# Autodesk Inventor assembly: MotorAssembly0
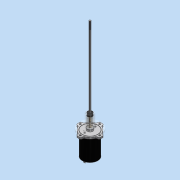
[picture p0: Inventor's stored thumbnail of the model, 180x180]
Saved by Autodesk Inventor 2017.3 (Build 213256000, 256)
## iProperties
Created: 2016-10-13
Part Number: MotorAssembly0
Document SubType Name: Assembly
Designer: techn
Author: techn
## Documents named in this file (7)
- G:\Projects\Submarine\Submarine-project\CAD\aft\MotorAssembly0.iam
- G:\Projects\Submarine\Submarine-project\CAD\aft\ShaftSeal\4mmShaftSeal.iam
- G:\Projects\Submarine\Submarine-project\CAD\aft\540DCMotor.ipt
- G:\Projects\Submarine\Submarine-project\CAD\aft\MotorMount.ipt
- G:\Projects\Submarine\Submarine-project\CAD\aft\MotorShaftCoupler.ipt
- G:\Projects\Submarine\Submarine-project\CAD\aft\DriveShaft4mm.ipt
- G:\Projects\Submarine\Submarine-project\CAD\aft\MotorMountNutHolder.ipt
## Components (6 placed, 6 different names)
1. 4mmShaftSeal:1 [sub-assembly] — Mate:3, Flush:1, Mate:7
2. 540DCMotor:1 — Mate:1, Mate:2, Mate:3, Mate:4, Mate:6
3. MotorMount:1 — Mate:1, Mate:4, Mate:5, Flush:1, Mate:6, Mate:9, Mate:10
4. MotorShaftCoupler:1 — Mate:2, Mate:5, Mate:8
5. DriveShaft4mm:1 — Mate:7, Mate:8
6. MotorMountNutHolder:1 — Mate:9, Mate:10, Angle:1
## Relationships (12: Mate 10, Flush 1, Angle 1)
- Mate:1: 540DCMotor:1 ↔ MotorMount:1
- Mate:2: 540DCMotor:1 ↔ MotorShaftCoupler:1
- Mate:3: 4mmShaftSeal:1 ↔ 540DCMotor:1
- Mate:4: 540DCMotor:1 ↔ MotorMount:1
- Mate:5 (1.27 mm): MotorMount:1 ↔ MotorShaftCoupler:1
- Flush:1: 4mmShaftSeal:1 ↔ MotorMount:1
- Mate:6: 540DCMotor:1 ↔ MotorMount:1
- Mate:7: 4mmShaftSeal:1 ↔ DriveShaft4mm:1
- Mate:8: MotorShaftCoupler:1 ↔ DriveShaft4mm:1
- Mate:9: MotorMount:1 ↔ MotorMountNutHolder:1
- Mate:10: MotorMount:1 ↔ MotorMountNutHolder:1
- Angle:1 (0 deg): MotorMountNutHolder:1
